# Autodesk Inventor assembly: assembly_caja
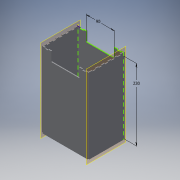
[picture p0: Inventor's stored thumbnail of the model, 180x180]
Saved by Autodesk Inventor 2019 (Build 230136000, 136)
## iProperties
Created: 2018-05-30
Part Number: assembly_caja
Document SubType Name: Assembly
Designer: seba
Author: seba
## Documents named in this file (5)
- C:\Users\seba\Documents\Inventor\intento_engranes2\assembly_caja.iam
- C:\Users\seba\Documents\Inventor\intento_engranes2\base_caja.ipt
- C:\Users\seba\Documents\Inventor\intento_engranes2\caja_lateral.ipt
- C:\Users\seba\Documents\Inventor\intento_engranes2\cara_posterior.ipt
- C:\Users\seba\Documents\Inventor\intento_engranes2\cara_superior.ipt
## Components (5 placed, 4 different names)
1. base_caja:1 — Mate:1, Mate:2, Mate:3, Mate:4, Mate:5, Mate:6, Mate:7
2. caja_lateral:1 — Mate:1, Mate:2, Mate:3, Mate:4, Mate:8, Mate:9, Mate:10
3. caja_lateral:2 — Mate:5, Mate:6, Mate:7, Mate:11
4. cara_posterior:1 — Mate:8, Mate:9, Mate:10, Mate:12, Mate:13, Mate:14
5. cara_superior:1 — Mate:11, Mate:12, Mate:13, Mate:14
## Relationships (14: Mate 14)
- Mate:1: base_caja:1 ↔ caja_lateral:1
- Mate:2: base_caja:1 ↔ caja_lateral:1
- Mate:3: base_caja:1 ↔ caja_lateral:1
- Mate:4: base_caja:1 ↔ caja_lateral:1
- Mate:5: base_caja:1 ↔ caja_lateral:2
- Mate:6: base_caja:1 ↔ caja_lateral:2
- Mate:7: base_caja:1 ↔ caja_lateral:2
- Mate:8: caja_lateral:1 ↔ cara_posterior:1
- Mate:9: caja_lateral:1 ↔ cara_posterior:1
- Mate:10: caja_lateral:1 ↔ cara_posterior:1
- Mate:11: caja_lateral:2 ↔ cara_superior:1
- Mate:12: cara_posterior:1 ↔ cara_superior:1
- Mate:13: cara_posterior:1 ↔ cara_superior:1
- Mate:14: cara_posterior:1 ↔ cara_superior:1
